# Autodesk Inventor assembly: PCB_Stack
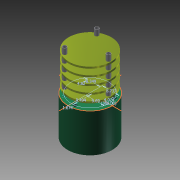
[picture p0: Inventor's stored thumbnail of the model, 180x180]
Saved by Autodesk Inventor 2011 SP2 (Build 150309200, 309)
## iProperties
Created: 2012-02-27
Part Number: PCB_Stack
Document SubType Name: Assembly
Designer: sungwook
Author: sungwook
## Documents named in this file (3)
- C:\Users\sungwook\Documents\Inventor\Micron20\Parts\Electronics\PCB_Stack.iam
- C:\Users\sungwook\Documents\Inventor\Micron20\Parts\Electronics\PCB_Post.iam
- C:\Users\sungwook\Documents\Inventor\Micron20\Parts\Electronics\Connector_PCB.ipt
## Components (6 placed, 2 different names)
1. PCB_Post:1 [sub-assembly] — Mate:1, Mate:2, Mate:3
2. PCB_Post:2 [sub-assembly] — Mate:1, Mate:2, Mate:3, Mate:4, Mate:5, Mate:6
3. PCB_Post:3 [sub-assembly] — Mate:7, Mate:8, Mate:9, Mate:10, Mate:11, Mate:12
4. PCB_Post:5 [sub-assembly] — Mate:10, Mate:11, Mate:12, Mate:14
5. PCB_Post:6 [sub-assembly] — Mate:4, Mate:5, Mate:6, Mate:7, Mate:8, Mate:9
6. Connector_PCB:1 — Mate:13, Angle:1, Mate:14
## Relationships (15: Mate 14, Angle 1)
- Mate:1: PCB_Post:1 ↔ PCB_Post:2
- Mate:2: PCB_Post:1 ↔ PCB_Post:2
- Mate:3: PCB_Post:1 ↔ PCB_Post:2
- Mate:4: PCB_Post:2 ↔ PCB_Post:6
- Mate:5: PCB_Post:2 ↔ PCB_Post:6
- Mate:6: PCB_Post:2 ↔ PCB_Post:6
- Mate:7: PCB_Post:3 ↔ PCB_Post:6
- Mate:8: PCB_Post:3 ↔ PCB_Post:6
- Mate:9: PCB_Post:3 ↔ PCB_Post:6
- Mate:10: PCB_Post:3 ↔ PCB_Post:5
- Mate:11: PCB_Post:3 ↔ PCB_Post:5
- Mate:12: PCB_Post:3 ↔ PCB_Post:5
- Mate:13: Connector_PCB:1
- Angle:1 (180 deg): Connector_PCB:1
- Mate:14 (3 mm): PCB_Post:5 ↔ Connector_PCB:1
